# Autodesk Inventor assembly: Full_Auto_Robot_Assembly_V1_15.10.25
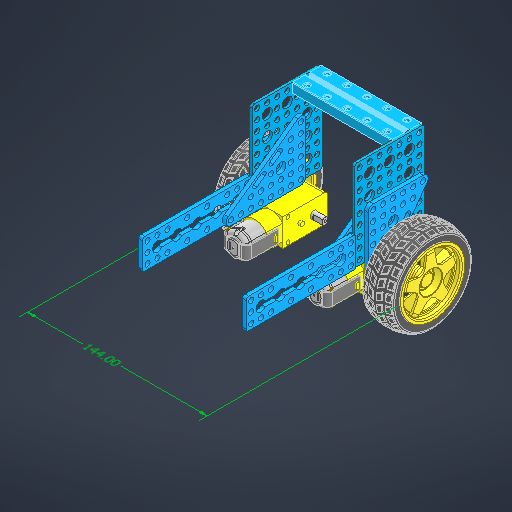
[picture p0: Inventor's stored thumbnail of the model, 512x512]
Saved by Autodesk Inventor 2026.1 (Build 301233020, 233B)
## iProperties
Created: 2025-10-11
Part Number: Full_Auto_Robot_Assembly_V1_15.10.25
Document SubType Name: Assembly
Designer: Asus
Author: Asus
## Documents named in this file (7)
- D:\KMITL\Computer_Programming\ComPro_Project\Robot_design_CAD_files\Full_Auto_Robot_Assembly_V1_15.10.25.iam
- D:\KMITL\Computer_Programming\ComPro_Project\Material_Parts_CAD_files\Metal_parts\Plate0324-088 V1.0.ipt
- D:\KMITL\Computer_Programming\ComPro_Project\Material_Parts_CAD_files\Metal_parts\Triangle Plate 6x8.ipt
- D:\KMITL\Computer_Programming\ComPro_Project\Material_Parts_CAD_files\Metal_parts\Beam0824-5.ipt
- D:\KMITL\Computer_Programming\ComPro_Project\Material_Parts_CAD_files\Metal_parts\Plate 7x9.ipt
- D:\KMITL\Computer_Programming\ComPro_Project\Material_Parts_CAD_files\Electronic_parts\yellow_dc_motor.ipt
- D:\KMITL\Computer_Programming\ComPro_Project\Material_Parts_CAD_files\Arudino_parts\Wheel D65x25.ipt
## Components (13 placed, 6 different names)
1. Plate0324-088 V1.0:1 — Rigid:4, Mate:1, Mate:2, Mate:3, Mate:15
2. Triangle Plate 6x8:1 — Rigid:4, Mate:1, Mate:2, Mate:3, Mate:4, Rigid:1
3. Beam0824-5:1 — Mate:6, Mate:7, Mate:8, Mate:11, Mate:12, Mate:13
4. Plate 7x9:1 — Mate:4, Rigid:1, Mate:5, Rigid:5, Mate:6, Mate:7, Mate:8
5. Triangle Plate 6x8:2 — Mate:5, Rigid:5, Mate:16
6. Plate0324-088 V1.0:2 — Rigid:6
7. Triangle Plate 6x8:3 — Rigid:6, Rotational:1, Mate:14
8. Plate 7x9:2 — Rotational:1, Mate:9, Mate:10, Rigid:7, Mate:11, Mate:12, Mate:13, Mate:14
9. Triangle Plate 6x8:4 — Mate:9, Mate:10, Rigid:7, Mate:17
10. yellow_dc_motor:1 — Mate:16, Rotational:2
11. yellow_dc_motor:2 — Mate:17, Rotational:3
12. Wheel D65x25:1 — Rotational:2
13. Wheel D65x25:2 — Rotational:3
## Relationships (25: Mate 17, WeldJoint 5, RevoluteJoint 3)
- Rigid:4 [WeldJoint]: Plate0324-088 V1.0:1 ↔ Triangle Plate 6x8:1
- Mate:1: Plate0324-088 V1.0:1 ↔ Triangle Plate 6x8:1
- Mate:2: Plate0324-088 V1.0:1 ↔ Triangle Plate 6x8:1
- Mate:3: Plate0324-088 V1.0:1 ↔ Triangle Plate 6x8:1
- Mate:4: Triangle Plate 6x8:1 ↔ Plate 7x9:1
- Rigid:1 [WeldJoint]: Triangle Plate 6x8:1 ↔ Plate 7x9:1
- Mate:5: Plate 7x9:1 ↔ Triangle Plate 6x8:2
- Rigid:5 [WeldJoint]: Plate 7x9:1 ↔ Triangle Plate 6x8:2
- Mate:6: Beam0824-5:1 ↔ Plate 7x9:1
- Mate:7: Beam0824-5:1 ↔ Plate 7x9:1
- Mate:8: Beam0824-5:1 ↔ Plate 7x9:1
- Rigid:6 [WeldJoint]: Plate0324-088 V1.0:2 ↔ Triangle Plate 6x8:3
- Rotational:1 [RevoluteJoint]: Triangle Plate 6x8:3 ↔ Plate 7x9:2
- Mate:9: Plate 7x9:2 ↔ Triangle Plate 6x8:4
- Mate:10: Plate 7x9:2 ↔ Triangle Plate 6x8:4
- Rigid:7 [WeldJoint]: Plate 7x9:2 ↔ Triangle Plate 6x8:4
- Mate:11: Beam0824-5:1 ↔ Plate 7x9:2
- Mate:12: Beam0824-5:1 ↔ Plate 7x9:2
- Mate:13: Beam0824-5:1 ↔ Plate 7x9:2
- Mate:14: Triangle Plate 6x8:3 ↔ Plate 7x9:2
- Mate:15: Plate0324-088 V1.0:1
- Mate:16: Triangle Plate 6x8:2 ↔ yellow_dc_motor:1
- Mate:17: Triangle Plate 6x8:4 ↔ yellow_dc_motor:2
- Rotational:2 [RevoluteJoint]: yellow_dc_motor:1 ↔ Wheel D65x25:1
- Rotational:3 [RevoluteJoint]: yellow_dc_motor:2 ↔ Wheel D65x25:2
